# Autodesk Inventor assembly: Passion-v2
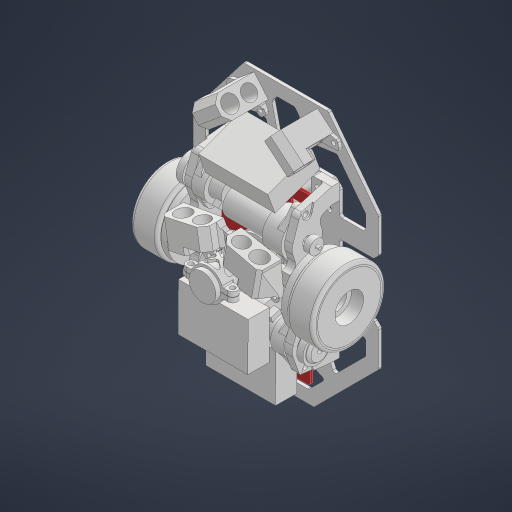
[picture p0: Inventor's stored thumbnail of the model, 512x512]
Saved by Autodesk Inventor 2023.5 (Build 275446000, 446)
## iProperties
Created: 2025-01-19
Part Number: Passion-v2
Document SubType Name: Assembly
Designer: IshiiLabHonda
Author: IshiiLabHonda
## Documents named in this file (28)
- C:\Users\IshiiLabHonda\Documents\Micromouse\Passion-v2\Inventor\Passion-v2-6\Passion-v2.iam
- C:\Users\IshiiLabHonda\Documents\Micromouse\Passion-v2\Inventor\Passion-v2-6\Origin\chassis.ipt
- C:\Users\IshiiLabHonda\Documents\Micromouse\Passion-v2\Inventor\Passion-v2-6\Readymade\Motor-8520.ipt
- C:\Users\IshiiLabHonda\Documents\Micromouse\Passion-v2\Inventor\Passion-v2-6\Readymade\Encoder-7S-400-2MC-50-00E.ipt
- C:\Users\IshiiLabHonda\Documents\Micromouse\Passion-v2\Inventor\Passion-v2-6\Readymade\Pinion-Gear_M0.3_15T.ipt
- C:\Users\IshiiLabHonda\Documents\Micromouse\Passion-v2\Inventor\Passion-v2-6\Readymade\Encoder-Gear_M0.3_29T.ipt
- C:\Users\IshiiLabHonda\Documents\Micromouse\Passion-v2\Inventor\Passion-v2-6\Readymade\Spur-Gear_M0.3_71T_t2.0_D8.ipt
- C:\Users\IshiiLabHonda\Documents\Micromouse\Passion-v2\Inventor\Passion-v2-6\Readymade\Wheel_MZH131W-N2.ipt
- C:\Users\IshiiLabHonda\Documents\Micromouse\Passion-v2\Inventor\Passion-v2-6\Readymade\Tire-MZW39-40.ipt
- C:\Users\IshiiLabHonda\Documents\Micromouse\Passion-v2\Inventor\Passion-v2-6\Readymade\Encoder-Gear-Spacer.ipt
- C:\Users\IshiiLabHonda\Documents\Micromouse\Passion-v2\Inventor\Passion-v2-6\Origin\motormount-r.ipt
- C:\Users\IshiiLabHonda\Documents\Micromouse\Passion-v2\Inventor\Passion-v2-6\Origin\motormount-l.ipt
- C:\Users\IshiiLabHonda\Documents\Micromouse\Passion-v2\Inventor\Passion-v2-6\Common\spacer-outwheel-m3-1.ipt
- C:\Users\IshiiLabHonda\Documents\Micromouse\Passion-v2\Inventor\Passion-v2-6\Origin\circuit.ipt
- C:\Users\IshiiLabHonda\Documents\Micromouse\Passion-v2\Inventor\Passion-v2-6\Origin\encodersupporter.ipt
- C:\Users\IshiiLabHonda\Documents\Micromouse\Passion-v2\Inventor\Passion-v2-6\Origin\sensormount.ipt
- C:\Users\IshiiLabHonda\Documents\Micromouse\Passion-v2\Inventor\Passion-v2-6\Origin\motorsupporter.ipt
- C:\Users\IshiiLabHonda\Documents\Micromouse\Passion-v2\Inventor\Passion-v2-6\Origin\sensorbase.ipt
- C:\Users\IshiiLabHonda\Documents\Micromouse\Passion-v2\Inventor\Passion-v2-6\Origin\frontsensorholder.ipt
- C:\Users\IshiiLabHonda\Documents\Micromouse\Passion-v2\Inventor\Passion-v2-6\Origin\fanmotor-mount-1.ipt
- C:\Users\IshiiLabHonda\Documents\Micromouse\Passion-v2\Inventor\Passion-v2-6\Origin\fanmotor-mount-2.ipt
- C:\Users\IshiiLabHonda\Documents\Micromouse\Passion-v2\Inventor\Passion-v2-6\Origin\fanmotor-mount-2-1.ipt
- C:\Users\IshiiLabHonda\Documents\Micromouse\Passion-v2\Inventor\Passion-v2-6\Origin\fan-concreate.ipt
- C:\Users\IshiiLabHonda\Documents\Micromouse\Passion-v2\Inventor\Passion-v2-6\Common\bearing_SMR63ZZ.ipt
- C:\Users\IshiiLabHonda\Documents\Micromouse\Passion-v2\Inventor\Passion-v2-6\Common\spacer_inwheel_1.1.ipt
- C:\Users\IshiiLabHonda\Documents\Micromouse\Passion-v2\Inventor\Passion-v2-6\Common\M3_bolt.ipt
- C:\Users\IshiiLabHonda\Documents\Micromouse\Passion-v2\Inventor\Passion-v2-6\Common\m2-5.5-spacer.ipt
- C:\Users\IshiiLabHonda\Documents\Micromouse\Passion-v2\Inventor\Passion-v2-6\Readymade\Lipo-1C-FX100C.ipt
## Components (45 placed, 27 different names)
1. chassis:1 — フラッシュ:1, メイト:1, メイト:2, メイト:71, メイト:82, メイト:115, メイト:122, メイト:135, メイト:136, メイト:137, メイト:138, メイト:139, メイト:140, メイト:141, メイト:142, メイト:186, メイト:188
2. Motor-8520:1 — メイト:12, メイト:87, メイト:156
3. Encoder-7S-400-2MC-50-00E:1 — メイト:13, メイト:61, フラッシュ:8
4. Pinion-Gear_M0.3_15T:1 — メイト:12, フラッシュ:7
5. Encoder-Gear_M0.3_29T:1 — メイト:13, メイト:18, メイト:19, フラッシュ:6
6. Spur-Gear_M0.3_71T_t2.0_D8:1 — メイト:17, メイト:59, フラッシュ:6, フラッシュ:7
7. Wheel_MZH131W-N2:1 — メイト:15, フラッシュ:2, メイト:17, メイト:56, メイト:59, メイト:60, メイト:143, メイト:144, メイト:145
8. Tire-MZW39-40:1 — メイト:15, フラッシュ:2
9. Encoder-Gear-Spacer:1 — メイト:18, メイト:19
10. motormount-r:1 — メイト:140, メイト:141, メイト:142, メイト:160, メイト:162, メイト:163, メイト:164, メイト:165, メイト:166, フラッシュ:9, メイト:167, メイト:168, メイト:170, メイト:178, メイト:180
11. Encoder-7S-400-2MC-50-00E:2 — メイト:34, メイト:65, フラッシュ:9
12. Motor-8520:2 — メイト:33, メイト:88, メイト:160, メイト:163
13. Spur-Gear_M0.3_71T_t2.0_D8:2 — メイト:29, フラッシュ:4, フラッシュ:5
14. Wheel_MZH131W-N2:2 — メイト:29, メイト:48
15. Tire-MZW39-40:2 — メイト:46
16. Pinion-Gear_M0.3_15T:2 — メイト:33, フラッシュ:4
17. Encoder-Gear_M0.3_29T:2 — メイト:34, フラッシュ:5
18. Encoder-Gear-Spacer:2
19. motormount-l:1 — メイト:137, メイト:138, メイト:139, メイト:143, メイト:152, メイト:154, メイト:155, メイト:156, メイト:157, メイト:158, メイト:159, フラッシュ:8, メイト:169, メイト:179
20. spacer-outwheel-m3-1:1 — メイト:46, メイト:48, メイト:167, メイト:168
21. Motor-8520:3 — メイト:82, メイト:100, メイト:101, メイト:125, メイト:130, メイト:132, メイト:134
22. circuit:1 — メイト:100, メイト:101, メイト:115, メイト:126, メイト:127, メイト:136, メイト:183, メイト:185, メイト:187, メイト:189, メイト:190, メイト:191
23. spacer-outwheel-m3-1:2 — メイト:56, メイト:60, メイト:148, メイト:152
24. encodersupporter:1 — メイト:61, メイト:157, メイト:158, メイト:159
25. encodersupporter:4 — メイト:65, メイト:164, メイト:165, メイト:166
26. sensormount:1 — メイト:71, メイト:122
27. motorsupporter:1 — メイト:87, メイト:154, メイト:155, メイト:179
28. motorsupporter:2 — メイト:88, メイト:162, メイト:180
29. frontsensorholder:1 — メイト:172, メイト:176, メイト:177, メイト:181
30. fanmotor-mount-1:1 — メイト:125, メイト:126, メイト:127
31. fanmotor-mount-2:1 — メイト:130, メイト:133, メイト:173, メイト:174
32. fanmotor-mount-2-1:1 — メイト:132, メイト:133
33. fan-concreate:1 — メイト:134, メイト:135
34. bearing_SMR63ZZ:1 — メイト:144, メイト:149, メイト:150, メイト:151
35. bearing_SMR63ZZ:2 — メイト:145, メイト:146, メイト:147, メイト:148
36. spacer_inwheel_1.1:1 — メイト:146, メイト:147, メイト:149
37. M3_bolt:1 — メイト:150, メイト:151
38. sensorbase:1 — メイト:169, メイト:170, メイト:172, メイト:173, メイト:174, メイト:176, メイト:177, メイト:178, メイト:181
39. m2-5.5-spacer:1 — メイト:183, メイト:190
40. m2-5.5-spacer:2 — メイト:185, メイト:191
41. m2-5.5-spacer:3 — メイト:186, メイト:187
42. m2-5.5-spacer:4 — メイト:188, メイト:189
43. Lipo-1C-FX100C:2
44. Lipo-1C-FX100C:3
45. Lipo-1C-FX100C:4
## Relationships (97: Mate 88, Flush 9)
- フラッシュ:1 [Flush]: chassis:1
- メイト:1 [Mate]: chassis:1
- メイト:2 [Mate]: chassis:1
- メイト:12 [Mate]: Motor-8520:1 ↔ Pinion-Gear_M0.3_15T:1
- メイト:13 [Mate]: Encoder-7S-400-2MC-50-00E:1 ↔ Encoder-Gear_M0.3_29T:1
- メイト:15 [Mate]: Wheel_MZH131W-N2:1 ↔ Tire-MZW39-40:1
- フラッシュ:2 [Flush]: Wheel_MZH131W-N2:1 ↔ Tire-MZW39-40:1
- メイト:17 [Mate]: Spur-Gear_M0.3_71T_t2.0_D8:1 ↔ Wheel_MZH131W-N2:1
- メイト:18 [Mate]: Encoder-Gear_M0.3_29T:1 ↔ Encoder-Gear-Spacer:1
- メイト:19 [Mate]: Encoder-Gear_M0.3_29T:1 ↔ Encoder-Gear-Spacer:1
- [Mate]: Wheel_MZH131W-N2:2 ↔ Tire-MZW39-40:2
- [Flush]: Wheel_MZH131W-N2:2 ↔ Tire-MZW39-40:2
- [Mate]: Spur-Gear_M0.3_71T_t2.0_D8:2 ↔ Wheel_MZH131W-N2:2
- メイト:29 [Mate]: Spur-Gear_M0.3_71T_t2.0_D8:2 ↔ Wheel_MZH131W-N2:2
- [Mate]: Encoder-Gear_M0.3_29T:2 ↔ Encoder-Gear-Spacer:2
- [Mate]: Encoder-Gear_M0.3_29T:2 ↔ Encoder-Gear-Spacer:2
- メイト:33 [Mate]: Motor-8520:2 ↔ Pinion-Gear_M0.3_15T:2
- メイト:34 [Mate]: Encoder-7S-400-2MC-50-00E:2 ↔ Encoder-Gear_M0.3_29T:2
- メイト:46 [Mate]: Tire-MZW39-40:2 ↔ spacer-outwheel-m3-1:1
- メイト:48 [Mate]: Wheel_MZH131W-N2:2 ↔ spacer-outwheel-m3-1:1
- フラッシュ:4 [Flush]: Spur-Gear_M0.3_71T_t2.0_D8:2 ↔ Pinion-Gear_M0.3_15T:2
- フラッシュ:5 [Flush]: Spur-Gear_M0.3_71T_t2.0_D8:2 ↔ Encoder-Gear_M0.3_29T:2
- メイト:56 [Mate]: Wheel_MZH131W-N2:1 ↔ spacer-outwheel-m3-1:2
- メイト:59 [Mate]: Spur-Gear_M0.3_71T_t2.0_D8:1 ↔ Wheel_MZH131W-N2:1
- メイト:60 [Mate]: Wheel_MZH131W-N2:1 ↔ spacer-outwheel-m3-1:2
- メイト:61 [Mate]: Encoder-7S-400-2MC-50-00E:1 ↔ encodersupporter:1
- メイト:65 [Mate]: Encoder-7S-400-2MC-50-00E:2 ↔ encodersupporter:4
- メイト:71 [Mate]: chassis:1 ↔ sensormount:1
- メイト:82 [Mate]: chassis:1 ↔ Motor-8520:3
- フラッシュ:6 [Flush]: Encoder-Gear_M0.3_29T:1 ↔ Spur-Gear_M0.3_71T_t2.0_D8:1
- フラッシュ:7 [Flush]: Pinion-Gear_M0.3_15T:1 ↔ Spur-Gear_M0.3_71T_t2.0_D8:1
- メイト:87 [Mate]: Motor-8520:1 ↔ motorsupporter:1
- メイト:88 [Mate]: Motor-8520:2 ↔ motorsupporter:2
- メイト:100 [Mate]: Motor-8520:3 ↔ circuit:1
- メイト:101 [Mate]: Motor-8520:3 ↔ circuit:1
- メイト:115 [Mate] (5.5 mm): chassis:1 ↔ circuit:1
- メイト:122 [Mate]: chassis:1 ↔ sensormount:1
- メイト:125 [Mate]: Motor-8520:3 ↔ fanmotor-mount-1:1
- メイト:126 [Mate]: circuit:1 ↔ fanmotor-mount-1:1
- メイト:127 [Mate]: circuit:1 ↔ fanmotor-mount-1:1
- メイト:130 [Mate]: Motor-8520:3 ↔ fanmotor-mount-2:1
- メイト:132 [Mate]: Motor-8520:3 ↔ fanmotor-mount-2-1:1
- メイト:133 [Mate]: fanmotor-mount-2:1 ↔ fanmotor-mount-2-1:1
- メイト:134 [Mate]: Motor-8520:3 ↔ fan-concreate:1
- メイト:135 [Mate] (0.5 mm): chassis:1 ↔ fan-concreate:1
- メイト:136 [Mate]: chassis:1 ↔ circuit:1
- メイト:137 [Mate]: chassis:1 ↔ motormount-l:1
- メイト:138 [Mate]: chassis:1 ↔ motormount-l:1
- メイト:139 [Mate]: chassis:1 ↔ motormount-l:1
- メイト:140 [Mate]: chassis:1 ↔ motormount-r:1
- メイト:141 [Mate]: chassis:1 ↔ motormount-r:1
- メイト:142 [Mate]: chassis:1 ↔ motormount-r:1
- メイト:143 [Mate]: Wheel_MZH131W-N2:1 ↔ motormount-l:1
- メイト:144 [Mate]: Wheel_MZH131W-N2:1 ↔ bearing_SMR63ZZ:1
- メイト:145 [Mate]: Wheel_MZH131W-N2:1 ↔ bearing_SMR63ZZ:2
- メイト:146 [Mate]: bearing_SMR63ZZ:2 ↔ spacer_inwheel_1.1:1
- メイト:147 [Mate]: bearing_SMR63ZZ:2 ↔ spacer_inwheel_1.1:1
- メイト:148 [Mate]: spacer-outwheel-m3-1:2 ↔ bearing_SMR63ZZ:2
- メイト:149 [Mate]: bearing_SMR63ZZ:1 ↔ spacer_inwheel_1.1:1
- メイト:150 [Mate]: bearing_SMR63ZZ:1 ↔ M3_bolt:1
- メイト:151 [Mate]: bearing_SMR63ZZ:1 ↔ M3_bolt:1
- メイト:152 [Mate]: motormount-l:1 ↔ spacer-outwheel-m3-1:2
- メイト:154 [Mate]: motormount-l:1 ↔ motorsupporter:1
- メイト:155 [Mate]: motormount-l:1 ↔ motorsupporter:1
- メイト:156 [Mate]: Motor-8520:1 ↔ motormount-l:1
- メイト:157 [Mate]: motormount-l:1 ↔ encodersupporter:1
- メイト:158 [Mate]: motormount-l:1 ↔ encodersupporter:1
- メイト:159 [Mate]: motormount-l:1 ↔ encodersupporter:1
- フラッシュ:8 [Flush]: Encoder-7S-400-2MC-50-00E:1 ↔ motormount-l:1
- メイト:160 [Mate]: motormount-r:1 ↔ Motor-8520:2
- メイト:162 [Mate]: motormount-r:1 ↔ motorsupporter:2
- メイト:163 [Mate]: motormount-r:1 ↔ Motor-8520:2
- メイト:164 [Mate]: motormount-r:1 ↔ encodersupporter:4
- メイト:165 [Mate]: motormount-r:1 ↔ encodersupporter:4
- メイト:166 [Mate]: motormount-r:1 ↔ encodersupporter:4
- フラッシュ:9 [Flush]: motormount-r:1 ↔ Encoder-7S-400-2MC-50-00E:2
- メイト:167 [Mate]: motormount-r:1 ↔ spacer-outwheel-m3-1:1
- メイト:168 [Mate]: motormount-r:1 ↔ spacer-outwheel-m3-1:1
- メイト:169 [Mate]: motormount-l:1 ↔ sensorbase:1
- メイト:170 [Mate]: motormount-r:1 ↔ sensorbase:1
- メイト:172 [Mate]: frontsensorholder:1 ↔ sensorbase:1
- メイト:173 [Mate]: fanmotor-mount-2:1 ↔ sensorbase:1
- メイト:174 [Mate]: fanmotor-mount-2:1 ↔ sensorbase:1
- メイト:176 [Mate]: frontsensorholder:1 ↔ sensorbase:1
- メイト:177 [Mate]: frontsensorholder:1 ↔ sensorbase:1
- メイト:178 [Mate]: motormount-r:1 ↔ sensorbase:1
- メイト:179 [Mate]: motormount-l:1 ↔ motorsupporter:1
- メイト:180 [Mate]: motormount-r:1 ↔ motorsupporter:2
- メイト:181 [Mate]: frontsensorholder:1 ↔ sensorbase:1
- メイト:183 [Mate]: circuit:1 ↔ m2-5.5-spacer:1
- メイト:185 [Mate]: circuit:1 ↔ m2-5.5-spacer:2
- メイト:186 [Mate]: chassis:1 ↔ m2-5.5-spacer:3
- メイト:187 [Mate]: circuit:1 ↔ m2-5.5-spacer:3
- メイト:188 [Mate]: chassis:1 ↔ m2-5.5-spacer:4
- メイト:189 [Mate]: circuit:1 ↔ m2-5.5-spacer:4
- メイト:190 [Mate]: circuit:1 ↔ m2-5.5-spacer:1
- メイト:191 [Mate]: circuit:1 ↔ m2-5.5-spacer:2
## Named parameters: d41_d25 = 0 mm, d42_d26 = 0 mm, d43_d28 = 0 mm, d46_d29 = 0 mm, d47_d30 = 0 mm
